# Autodesk Inventor assembly: Hauptteil
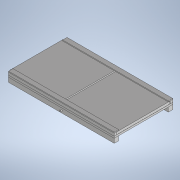
[picture p0: Inventor's stored thumbnail of the model, 180x180]
Saved by Autodesk Inventor 2020.3 (Build 243373000, 373)
## iProperties
Created: 2020-09-30
Part Number: Hauptteil
Document SubType Name: Assembly
Designer: Mara
Author: Mara
## Documents named in this file (6)
- C:\Users\Mara\Masterarbeit_CAD\Rampe\Hauptteil.iam
- C:\Users\Mara\Masterarbeit_CAD\Rampe\o_lange_Stange.ipt
- C:\Users\Mara\Masterarbeit_CAD\Rampe\u_lange_Stange.ipt
- C:\Users\Mara\Masterarbeit_CAD\Rampe\o_fache_Stange.ipt
- C:\Users\Mara\Masterarbeit_CAD\Rampe\o_grosses_Brett.ipt
- C:\Users\Mara\Masterarbeit_CAD\Rampe\o_Einlegplatten.ipt
## Components (9 placed, 5 different names)
1. o_lange_Stange:1 — Mate:2, Flush:3, Flush:4, Mate:4, Flush:5, Flush:6, Mate:9, Mate:10, Flush:15
2. u_lange_Stange:1 — Mate:11, Flush:13, Flush:14
3. o_fache_Stange:1 — Mate:3, Flush:7, Flush:8
4. o_grosses_Brett:1 — Mate:1, Flush:1, Flush:2, Mate:2, Flush:3, Flush:4, Mate:7, Mate:8, Mate:11, Flush:13, Flush:14, Mate:12, Flush:16
5. o_fache_Stange:2 — Mate:4, Flush:5, Flush:6
6. o_lange_Stange:2 — Mate:1, Flush:1, Flush:2, Mate:3, Flush:7, Flush:8
7. u_lange_Stange:2 — Mate:12, Flush:15, Flush:16
8. o_Einlegplatten:1 — Mate:7, Mate:9
9. o_Einlegplatten:2 — Mate:8, Mate:10
## Relationships (22: Flush 12, Mate 10)
- Mate:1: o_grosses_Brett:1 ↔ o_lange_Stange:2
- Flush:1: o_grosses_Brett:1 ↔ o_lange_Stange:2
- Flush:2: o_grosses_Brett:1 ↔ o_lange_Stange:2
- Mate:2: o_lange_Stange:1 ↔ o_grosses_Brett:1
- Flush:3: o_lange_Stange:1 ↔ o_grosses_Brett:1
- Flush:4: o_lange_Stange:1 ↔ o_grosses_Brett:1
- Mate:3: o_fache_Stange:1 ↔ o_lange_Stange:2
- Mate:4: o_lange_Stange:1 ↔ o_fache_Stange:2
- Flush:5: o_lange_Stange:1 ↔ o_fache_Stange:2
- Flush:6: o_lange_Stange:1 ↔ o_fache_Stange:2
- Flush:7: o_fache_Stange:1 ↔ o_lange_Stange:2
- Flush:8: o_fache_Stange:1 ↔ o_lange_Stange:2
- Mate:7: o_grosses_Brett:1 ↔ o_Einlegplatten:1
- Mate:8: o_grosses_Brett:1 ↔ o_Einlegplatten:2
- Mate:9 (2 mm): o_lange_Stange:1 ↔ o_Einlegplatten:1
- Mate:10 (2 mm): o_lange_Stange:1 ↔ o_Einlegplatten:2
- Mate:11: u_lange_Stange:1 ↔ o_grosses_Brett:1
- Flush:13: u_lange_Stange:1 ↔ o_grosses_Brett:1
- Flush:14: u_lange_Stange:1 ↔ o_grosses_Brett:1
- Mate:12: o_grosses_Brett:1 ↔ u_lange_Stange:2
- Flush:15: o_lange_Stange:1 ↔ u_lange_Stange:2
- Flush:16: o_grosses_Brett:1 ↔ u_lange_Stange:2
